# Autodesk Inventor assembly: postAssembly
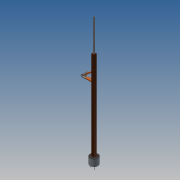
[picture p0: Inventor's stored thumbnail of the model, 180x180]
Saved by Autodesk Inventor 2014 SP1 (Build 180222100, 222)
## iProperties
Created: 2013-12-02
Part Number: postAssembly
Document SubType Name: Assembly
Designer: Dave
Author: Dave
## Documents named in this file (8)
- C:\Users\Dave\Desktop\hera-cad\support\postAssembly.iam
- C:\Users\Dave\Desktop\hera-cad\support\postSonotube.ipt
- C:\Users\Dave\Desktop\hera-cad\support\postRebar.ipt
- C:\Users\Dave\Desktop\hera-cad\support\post.ipt
- C:\Users\Dave\Desktop\hera-cad\support\postExtender.ipt
- C:\Users\Dave\Desktop\hera-cad\support\postCement.ipt
- C:\Users\Dave\Desktop\hera-cad\support\heightMarker.ipt
- C:\Users\Dave\Desktop\hera-cad\support\postStandSupport.iam
## Components (9 placed, 7 different names)
1. postSonotube:1 — Insert:1, Insert:3
2. post:1 — Insert:1, Insert:2, Mate:8, Mate:9, Flush:1
3. postExtender:1 — Insert:2
4. postCement:1 — Insert:3
5. heightMarker:1 — Mate:8, Mate:10
6. postStandSupport:1 [sub-assembly] — Mate:9, Flush:1, Mate:10
7. postRebar:1
8. postRebar:2
9. postRebar:3
## Component patterns: rebar (3 elements)
## Relationships (7: Insert 3, Mate 3, Flush 1)
- Insert:1: postSonotube:1 ↔ post:1
- Insert:2: post:1 ↔ postExtender:1
- Insert:3: postSonotube:1 ↔ postCement:1
- Mate:8 (-1143.61 mm): post:1 ↔ heightMarker:1
- Mate:9: post:1 ↔ postStandSupport:1
- Flush:1: post:1 ↔ postStandSupport:1
- Mate:10 (1553.464 mm): heightMarker:1 ↔ postStandSupport:1
